# Autodesk Inventor assembly: Ensamblaje2
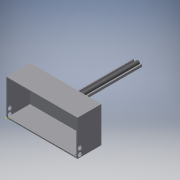
[picture p0: Inventor's stored thumbnail of the model, 180x180]
Saved by Autodesk Inventor 2017 (Build 210142000, 142)
## iProperties
Part Number: Ensamblaje2
Material: Genérico
Document SubType Name: Assembly
Designer: diego
Author: diego
## Documents named in this file (6)
- E:\inventor 2017\Ensamblaje2.iam
- E:\inventor 2017\Pieza2.ipt
- E:\inventor 2017\Pieza3.ipt
- E:\inventor 2017\Pieza4.ipt
- E:\inventor 2017\Pieza5.ipt
- E:\inventor 2017\Pieza6.ipt
## Components (5 placed, 5 different names)
1. Pieza2:1 — De rotación:1
2. Pieza3:1 — De rotación:1, Rígido:1, Rígido:2, De rotación:2
3. Pieza4:1 — Rígido:1
4. Pieza5:1 — Rígido:2
5. Pieza6:1 — De rotación:2
## Relationships (4: RevoluteJoint 2, WeldJoint 2)
- De rotación:1 [RevoluteJoint]: Pieza2:1 ↔ Pieza3:1
- Rígido:1 [WeldJoint]: Pieza3:1 ↔ Pieza4:1
- Rígido:2 [WeldJoint]: Pieza3:1 ↔ Pieza5:1
- De rotación:2 [RevoluteJoint]: Pieza3:1 ↔ Pieza6:1
